# Autodesk Inventor assembly: Head_V3_Assembly
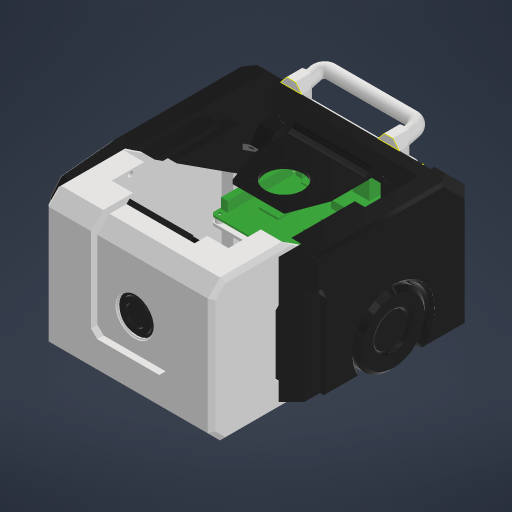
[picture p0: Inventor's stored thumbnail of the model, 512x512]
Saved by Autodesk Inventor 2024 (Build 280153000, 153)
## iProperties
Created: 2025-09-25
Part Number: Head_V3_Assembly
Document SubType Name: Assembly
Designer: kevin
Author: kevin
## Documents named in this file (14)
- C:\Users\kevin\Desktop\SeniorDesign\Head_V3\Head_V3_Assembly.iam
- C:\Users\kevin\Desktop\SeniorDesign\Emeet_Camera.ipt
- C:\Users\kevin\Desktop\SeniorDesign\Head_V3\Head_base_mount.ipt
- C:\Users\kevin\Desktop\SeniorDesign\Head_V3\Camera_Clip.ipt
- C:\Users\kevin\Desktop\SeniorDesign\Head_V3\RaspberryPi_Encloser.iam
- C:\Users\kevin\Desktop\SeniorDesign\Head_V3\Head_Left_Panel.ipt
- C:\Users\kevin\Desktop\SeniorDesign\Head_V3\Head_Right_Panel.ipt
- C:\Users\kevin\Desktop\SeniorDesign\Head_V3\Head_Backplate.ipt
- C:\Users\kevin\Desktop\SeniorDesign\Head_V3\Fan.ipt
- C:\Users\kevin\Desktop\SeniorDesign\Head_V3\Head_Top.ipt
- C:\Users\kevin\Desktop\SeniorDesign\Head_V3\Head_Handle.ipt
- C:\Users\kevin\Desktop\SeniorDesign\Head_V3\Head_Fin.ipt
- C:\Users\kevin\Desktop\SeniorDesign\Head_V3\Head_Fin_Bottom.ipt
- C:\Users\kevin\Desktop\SeniorDesign\Head_V3\Esp32_Holder.ipt
## Components (13 placed, 13 different names)
1. Emeet_Camera:1 — Flush:1, Mate:1, Flush:2, Flush:3, Flush:6, Flush:7
2. Head_base_mount:1 — Mate:1, Flush:2, Flush:3, Flush:6, Flush:7, Mate:2, Flush:8, Flush:9, Flush:10, Mate:3, Flush:11, Mate:6, Flush:24
3. Camera_Clip:1 — Mate:2, Flush:8, Flush:9
4. RaspberryPi_Encloser:1 [sub-assembly]
5. Head_Left_Panel:1 — Flush:10, Flush:12, Flush:13, Symmetry:2
6. Head_Right_Panel:1 — Mate:3, Flush:11, Flush:12, Flush:15, Symmetry:2
7. Head_Backplate:1 — Flush:14, Mate:5
8. Fan:1 — Mate:5, Mate:6
9. Head_Top:1 — Flush:16, Flush:17, Flush:18, Flush:19, Flush:20, Flush:21, Flush:22
10. Head_Handle:1 — Flush:18, Flush:19, Flush:20
11. Head_Fin:1 — Flush:21, Flush:22
12. Head_Fin_Bottom:1 — Flush:23
13. Esp32_Holder:1 — Flush:24
## Relationships (29: Flush 22, Mate 5, Symmetry 2)
- Flush:1 (0.2 mm): Emeet_Camera:1
- Mate:1: Emeet_Camera:1 ↔ Head_base_mount:1
- Flush:2: Emeet_Camera:1 ↔ Head_base_mount:1
- Flush:3: Emeet_Camera:1 ↔ Head_base_mount:1
- Flush:6 (0.2032 mm): Emeet_Camera:1 ↔ Head_base_mount:1
- Flush:7: Emeet_Camera:1 ↔ Head_base_mount:1
- Mate:2: Head_base_mount:1 ↔ Camera_Clip:1
- Flush:8: Head_base_mount:1 ↔ Camera_Clip:1
- Flush:9: Head_base_mount:1 ↔ Camera_Clip:1
- Flush:10: Head_base_mount:1 ↔ Head_Left_Panel:1
- Mate:3: Head_base_mount:1 ↔ Head_Right_Panel:1
- Flush:11: Head_base_mount:1 ↔ Head_Right_Panel:1
- Flush:12: Head_Left_Panel:1 ↔ Head_Right_Panel:1
- Flush:13 (0.2 mm): Head_Left_Panel:1
- Flush:14: Head_Backplate:1
- Flush:15 (0.2 mm): Head_Right_Panel:1
- Mate:5 (0.5 mm): Head_Backplate:1 ↔ Fan:1
- Mate:6 (0.5 mm): Head_base_mount:1 ↔ Fan:1
- Flush:16: Head_Top:1
- Symmetry:1
- Flush:17: Head_Top:1
- Flush:18: Head_Top:1 ↔ Head_Handle:1
- Flush:19: Head_Top:1 ↔ Head_Handle:1
- Flush:20: Head_Top:1 ↔ Head_Handle:1
- Flush:21: Head_Top:1 ↔ Head_Fin:1
- Flush:22: Head_Top:1 ↔ Head_Fin:1
- Flush:23: Head_Fin_Bottom:1
- Symmetry:2: Head_Left_Panel:1 ↔ Head_Right_Panel:1
- Flush:24: Head_base_mount:1 ↔ Esp32_Holder:1
